# Autodesk Inventor assembly: om_Interior
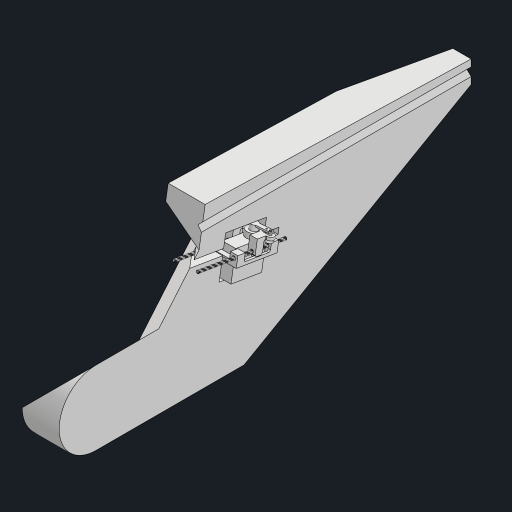
[picture p0: Inventor's stored thumbnail of the model, 512x512]
Saved by Autodesk Inventor 2023 (Build 270158000, 158)
## iProperties
Created: 2022-06-21
Part Number: om_Interior
Document SubType Name: Assembly
Designer: legot
Author: legot
## Documents named in this file (3)
- C:\Users\legot\OneDrive\ドキュメント\Inventor\HIKOSAPO\OM\om_Interior.iam
- C:\Users\legot\OneDrive\ドキュメント\Inventor\HIKOSAPO\OM\om_Body.ipt
- C:\Users\legot\OneDrive\ドキュメント\Inventor\HIKOSAPO\DropMechanism\om_Drop.iam
## Components (2 placed, 2 different names)
1. om_Body:1 — メイト:9, メイト:11, メイト:12
2. om_Drop:1 [sub-assembly] — メイト:9, メイト:11, メイト:12
## Relationships (3: Mate 3)
- メイト:9 [Mate]: om_Body:1 ↔ om_Drop:1
- メイト:11 [Mate]: om_Body:1 ↔ om_Drop:1
- メイト:12 [Mate]: om_Body:1 ↔ om_Drop:1
